# Autodesk Inventor assembly: Assembly1
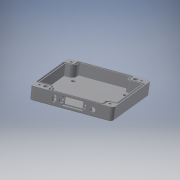
[picture p0: Inventor's stored thumbnail of the model, 180x180]
Saved by Autodesk Inventor 2018 (Build 220112000, 112)
## iProperties
Created: 2018-04-13
Part Number: Assembly1
Document SubType Name: Assembly
Designer: Hogar
Author: Hogar
## Documents named in this file (2)
- C:\Users\Hogar\Documents\SS\DVI\Isometric.iam
- C:\Users\Hogar\Documents\SS\ECDL OCR\5500-37 LID.ipt
## Components (1 placed, 1 different names)
1. 5500-37 LID:1 — Flush:1
## Relationships (1: Flush 1)
- Flush:1: 5500-37 LID:1
